# Autodesk Inventor assembly: Single Acting Piston_MIR
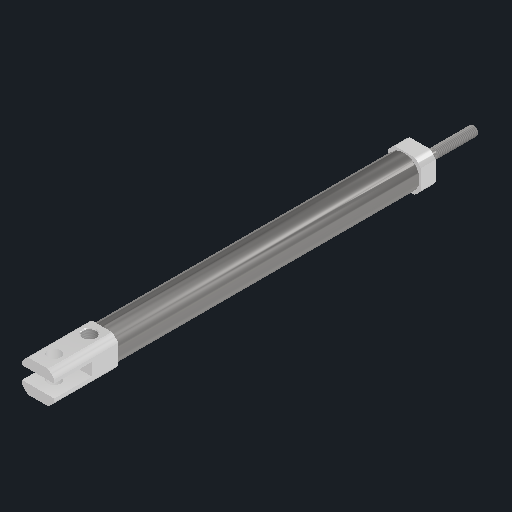
[picture p0: Inventor's stored thumbnail of the model, 512x512]
Saved by Autodesk Inventor 2024 (Build 280153000, 153)
## iProperties
Created: 2022-09-23
Part Number: Single Acting Piston_MIR
Document SubType Name: Assembly
Designer: avere
Mass: 12.2112 g
Surface Area: 100.21 cm^2
Volume: 12.2112 cm^3
Author: maxxw
## Documents named in this file (3)
- C:\Users\avere\Documents\rbp_cad\zoomba_v0.3\chassis\mirrored_parts\Single Acting Piston_MIR.iam
- C:\Users\avere\Documents\rbp_cad\zoomba_v0.3\chassis\mirrored_parts\Single Acting Piston Rod_MIR.ipt
- C:\Users\avere\Documents\rbp_cad\zoomba_v0.3\chassis\mirrored_parts\Single Acting Piston Body_MIR.ipt
## Components (2 placed, 2 different names)
1. Single Acting Piston Rod_MIR:1 — Mate:2, Mate:1
2. Single Acting Piston Body_MIR:1 — Mate:2, Mate:1
## Relationships (2: Mate 2)
- Mate:2: Single Acting Piston Rod_MIR:1 ↔ Single Acting Piston Body_MIR:1
- Mate:1: Single Acting Piston Rod_MIR:1 ↔ Single Acting Piston Body_MIR:1
